# Autodesk Inventor assembly: Core
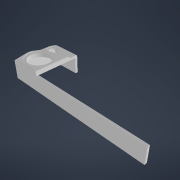
[picture p0: Inventor's stored thumbnail of the model, 180x180]
Saved by Autodesk Inventor 2022 (Build 260153000, 153)
## iProperties
Created: 2022-04-08
Part Number: Core
Document SubType Name: Assembly
Designer: Kalugin_a
Author: Kalugin_a
## Documents named in this file (6)
- D:\GitHUB\MELAS\Workspace\BoordyaBeatBox\Core.iam
- D:\GitHUB\MELAS\Workspace\BoordyaBeatBox\Front_L.ipt
- D:\GitHUB\MELAS\Workspace\BoordyaBeatBox\Front1.ipt
- D:\GitHUB\MELAS\Workspace\BoordyaBeatBox\Top.ipt
- D:\GitHUB\MELAS\Workspace\BoordyaBeatBox\side.ipt
- D:\GitHUB\MELAS\Workspace\BoordyaBeatBox\bottom.ipt
## Components (5 placed, 5 different names)
1. Front_L:1 — Совмещение:1, Совмещение:2, Совмещение:3, Совмещение:4, Совмещение:5, Совмещение:7
2. Front1:1 — Совмещение:1, Совмещение:2
3. Top:1 — Совмещение:3, Совмещение:4, Совмещение:6
4. side:1 — Совмещение:5, Совмещение:6, Совмещение:8
5. bottom:1 — Совмещение:7, Совмещение:8
## Relationships (8: Mate 8)
- Совмещение:1 [Mate]: Front_L:1 ↔ Front1:1
- Совмещение:2 [Mate]: Front_L:1 ↔ Front1:1
- Совмещение:3 [Mate]: Front_L:1 ↔ Top:1
- Совмещение:4 [Mate]: Front_L:1 ↔ Top:1
- Совмещение:5 [Mate]: Front_L:1 ↔ side:1
- Совмещение:6 [Mate]: Top:1 ↔ side:1
- Совмещение:7 [Mate]: Front_L:1 ↔ bottom:1
- Совмещение:8 [Mate]: side:1 ↔ bottom:1
